# Autodesk Inventor assembly: Assembly1
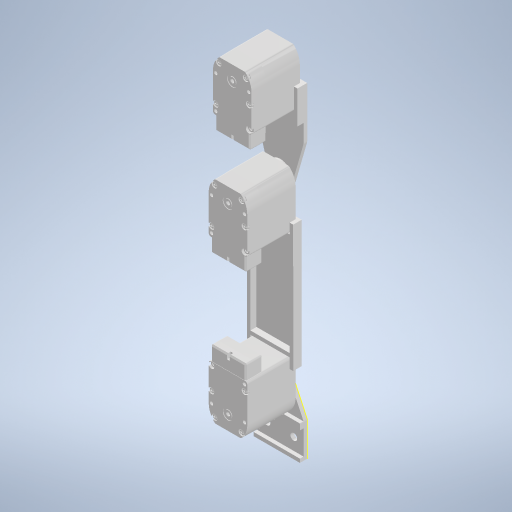
[picture p0: Inventor's stored thumbnail of the model, 512x512]
Saved by Autodesk Inventor 2024.3 (Build 283343000, 343)
## iProperties
Created: 2024-11-22
Part Number: Assembly1
Document SubType Name: Assembly
Designer: azara
Author: azara
## Documents named in this file (5)
- C:\Users\azara\Documents\kondo-PMX-scara-robot-arm\Assembly1.iam
- C:\Users\azara\Documents\kondo-PMX-scara-robot-arm\robot-arm-frame-base.ipt
- C:\Users\azara\Documents\kondo-PMX-scara-robot-arm\kondo-PMX-9200_scale.ipt
- C:\Users\azara\Documents\kondo-PMX-scara-robot-arm\robot-arm-frame.ipt
- C:\Users\azara\Documents\kondo-PMX-scara-robot-arm\robot-arm-frame-output.ipt
## Components (6 placed, 4 different names)
1. robot-arm-frame:1 — 挿入:3, 挿入:4, 挿入:5, 挿入:6
2. kondo-PMX-9200_scale:1 — 挿入:3, 挿入:4, 挿入:11
3. kondo-PMX-9200_scale:2 — 挿入:5, 挿入:6, 挿入:12
4. kondo-PMX-9200_scale:3 — 挿入:7, 挿入:8
5. robot-arm-frame-output:1 — 挿入:7, 挿入:8, 挿入:12
6. robot-arm-frame-base:1 — 挿入:11
## Relationships (8: Insert 8)
- 挿入:3 [Insert]: robot-arm-frame:1 ↔ kondo-PMX-9200_scale:1
- 挿入:4 [Insert]: robot-arm-frame:1 ↔ kondo-PMX-9200_scale:1
- 挿入:5 [Insert]: robot-arm-frame:1 ↔ kondo-PMX-9200_scale:2
- 挿入:6 [Insert]: robot-arm-frame:1 ↔ kondo-PMX-9200_scale:2
- 挿入:7 [Insert]: kondo-PMX-9200_scale:3 ↔ robot-arm-frame-output:1
- 挿入:8 [Insert]: kondo-PMX-9200_scale:3 ↔ robot-arm-frame-output:1
- 挿入:11 [Insert] (5.9 mm): kondo-PMX-9200_scale:1 ↔ robot-arm-frame-base:1
- 挿入:12 [Insert] (5.9 mm): kondo-PMX-9200_scale:2 ↔ robot-arm-frame-output:1
